# Autodesk Inventor assembly: Intake New Robot
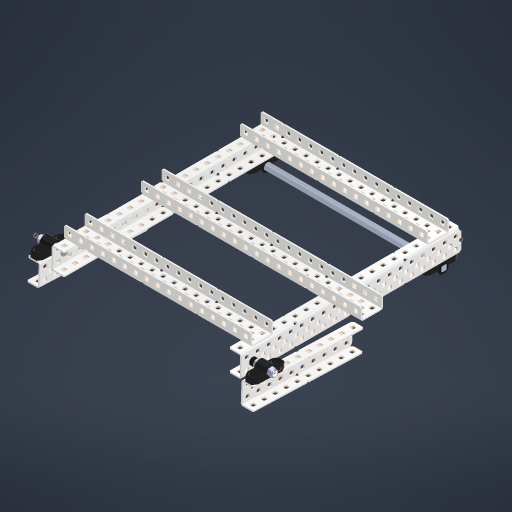
[picture p0: Inventor's stored thumbnail of the model, 512x512]
Saved by Autodesk Inventor 2023 (Build 270158000, 158)
## iProperties
Created: 2023-11-27
Part Number: Intake New Robot
Document SubType Name: Assembly
Designer: Robodox
Author: Robodox
## Documents named in this file (17)
- C:\Users\diego\OneDrive\Documents\GitHub\2023-599Z\BBotCAD\Intake New Robot.iam
- C:\Users\diego\OneDrive\Documents\GitHub\2023-599Z\BBotCAD\VEX-CAD-Inventor-1.4.0\Structure\C Channel\Aluminum 1x2x1\Alu C 1x2x1x10.ipt
- C:\Users\diego\OneDrive\Documents\GitHub\2023-599Z\BBotCAD\VEX-CAD-Inventor-1.4.0\Structure\Hardware\Screw Steel - Star\SScrew Star Smooth 1.000.ipt
- C:\Users\Robodox\Documents\GitHub\2023-599Z\BBotCAD\VEX-CAD-Inventor-1.4.0\Structure\Hardware\Screw Steel - Star.ipt
- C:\Users\diego\OneDrive\Documents\GitHub\2023-599Z\BBotCAD\VEX-CAD-Inventor-1.4.0\Structure\Hardware\Nut Nylock.ipt
- C:\Users\diego\OneDrive\Documents\GitHub\2023-599Z\BBotCAD\VEX-CAD-Inventor-1.4.0\Structure\Hardware\Nut Keps.ipt
- C:\Users\diego\OneDrive\Documents\GitHub\2023-599Z\BBotCAD\VEX-CAD-Inventor-1.4.0\Motion\Spacers\Spacer Plastic\PSpacer 4.6.ipt
- C:\Users\Robodox\Documents\GitHub\2023-599Z\BBotCAD\VEX-CAD-Inventor-1.4.0\Motion\Spacers\Spacer Plastic.ipt
- C:\Users\diego\OneDrive\Documents\GitHub\2023-599Z\BBotCAD\VEX-CAD-Inventor-1.4.0\Structure\C Channel\Aluminum 1x2x1\Alu C 1x2x1x20.ipt
- C:\Users\diego\OneDrive\Documents\GitHub\2023-599Z\BBotCAD\VEX-CAD-Inventor-1.4.0\Structure\C Channel\Aluminum 1x2x1\Alu C 1x2x1x1.ipt
- C:\Users\diego\OneDrive\Documents\GitHub\2023-599Z\BBotCAD\VEX-CAD-Inventor-1.4.0\Motion\Shaft HS\HS Pillow Bearing Block.ipt
- C:\Users\diego\OneDrive\Documents\GitHub\2023-599Z\BBotCAD\VEX-CAD-Inventor-1.4.0\Motion\Shaft HS\HS Spacer\HSpacer .0625.ipt
- C:\Users\diego\OneDrive\Documents\GitHub\2023-599Z\BBotCAD\VEX-CAD-Inventor-1.4.0\Motion\Shaft HS\HS Spacer.ipt
- C:\Users\diego\OneDrive\Documents\GitHub\2024-599Z\2024-599Z\Cad\VEX-CAD-Inventor-1.4.0\Structure\C Channel\Aluminum 1x2x1\Alu C 1x2x1x17.ipt
- C:\Users\diego\OneDrive\Documents\GitHub\2024-599Z\2024-599Z\Cad\VEX-CAD-Inventor-1.4.0\Structure\C Channel\Aluminum 1x2x1\Alu C 1x2x1x20.ipt
- C:\Users\diego\OneDrive\Documents\GitHub\2024-599Z\2024-599Z\Cad\VEX-CAD-Inventor-1.4.0\Motion\Shaft HS\Shaft HS\Shaft HS 8.5 in.ipt
- C:\Users\diego\OneDrive\Documents\GitHub\2024-599Z\2024-599Z\Cad\VEX-CAD-Inventor-1.4.0\Motion\Shaft HS\Shaft HS.ipt
## Components (24 placed, 11 different names)
1. Alu C 1x2x1x10:1 — Insert:24, Insert:25
2. Alu C 1x2x1x10:2 — Insert:26, Insert:27
3. SScrew Star Smooth 1.000:1 — Insert:5, Insert:21, Insert:23, Insert:35
4. Nut Nylock:1 — Insert:23
5. Nut Nylock:2 — Insert:15
6. Nut Keps:2 — Insert:13, Mate:5
7. PSpacer 4.6:1 — Insert:21, Insert:22
8. Alu C 1x2x1x20:2 — Insert:5, Insert:30, Insert:33, Insert:37, Insert:38, Insert:40, Mate:16, Insert:42, Insert:43
9. Nut Keps:3 — Insert:22
10. Alu C 1x2x1x1:1 — Insert:14, Mate:4
11. Alu C 1x2x1x20:4 — Insert:11, Insert:12, Insert:29, Insert:34, Insert:36, Insert:39, Insert:41, Insert:44
12. SScrew Star Smooth 1.000:2 — Insert:11, Insert:14, Insert:15
13. PSpacer 4.6:2 — Insert:12, Insert:13
14. HS Pillow Bearing Block:1 — Insert:26, Insert:27, Mate:4, Mate:5
15. HS Pillow Bearing Block:2 — Insert:24, Insert:25, Mate:14, Mate:15
16. HS Pillow Bearing Block:3 — Insert:30, Insert:33, Mate:18
17. HS Pillow Bearing Block:4 — Insert:29, Insert:34
18. HSpacer .0625:1 — Insert:47, Mate:18
19. Alu C 1x2x1x1:2 — Insert:35, Mate:14, Mate:15
20. Alu C 1x2x1x17:1 — Insert:36, Insert:37, Insert:38, Insert:39
21. Alu C 1x2x1x17:2 — Insert:40, Insert:41
22. HSpacer .0625:2 — Insert:46
23. Alu C 1x2x1x20:5 — Mate:16, Insert:42, Insert:43, Insert:44
24. Shaft HS 8.5 in:1 — Insert:46, Insert:47
## Relationships (35: Insert 29, Mate 6)
- Insert:5: SScrew Star Smooth 1.000:1 ↔ Alu C 1x2x1x20:2
- Insert:11: Alu C 1x2x1x20:4 ↔ SScrew Star Smooth 1.000:2
- Insert:12: Alu C 1x2x1x20:4 ↔ PSpacer 4.6:2
- Insert:13: Nut Keps:2 ↔ PSpacer 4.6:2
- Insert:14 (-15.494 mm): Alu C 1x2x1x1:1 ↔ SScrew Star Smooth 1.000:2
- Insert:15 (-3.048 mm): Nut Nylock:2 ↔ SScrew Star Smooth 1.000:2
- Insert:21 (-23.8252 mm): SScrew Star Smooth 1.000:1 ↔ PSpacer 4.6:1
- Insert:22: PSpacer 4.6:1 ↔ Nut Keps:3
- Insert:23 (-3.048 mm): SScrew Star Smooth 1.000:1 ↔ Nut Nylock:1
- Insert:24: Alu C 1x2x1x10:1 ↔ HS Pillow Bearing Block:2
- Insert:25: Alu C 1x2x1x10:1 ↔ HS Pillow Bearing Block:2
- Insert:26: Alu C 1x2x1x10:2 ↔ HS Pillow Bearing Block:1
- Insert:27: Alu C 1x2x1x10:2 ↔ HS Pillow Bearing Block:1
- Mate:4: Alu C 1x2x1x1:1 ↔ HS Pillow Bearing Block:1
- Mate:5: Nut Keps:2 ↔ HS Pillow Bearing Block:1
- Insert:29: Alu C 1x2x1x20:4 ↔ HS Pillow Bearing Block:4
- Insert:30: Alu C 1x2x1x20:2 ↔ HS Pillow Bearing Block:3
- Insert:33: Alu C 1x2x1x20:2 ↔ HS Pillow Bearing Block:3
- Insert:34: Alu C 1x2x1x20:4 ↔ HS Pillow Bearing Block:4
- Insert:35 (8.382 mm): SScrew Star Smooth 1.000:1 ↔ Alu C 1x2x1x1:2
- Mate:14: HS Pillow Bearing Block:2 ↔ Alu C 1x2x1x1:2
- Mate:15: HS Pillow Bearing Block:2 ↔ Alu C 1x2x1x1:2
- Insert:36: Alu C 1x2x1x20:4 ↔ Alu C 1x2x1x17:1
- Insert:37: Alu C 1x2x1x20:2 ↔ Alu C 1x2x1x17:1
- Insert:38: Alu C 1x2x1x20:2 ↔ Alu C 1x2x1x17:1
- Insert:39: Alu C 1x2x1x20:4 ↔ Alu C 1x2x1x17:1
- Insert:40: Alu C 1x2x1x20:2 ↔ Alu C 1x2x1x17:2
- Insert:41: Alu C 1x2x1x20:4 ↔ Alu C 1x2x1x17:2
- Mate:16: Alu C 1x2x1x20:2 ↔ Alu C 1x2x1x20:5
- Insert:42: Alu C 1x2x1x20:2 ↔ Alu C 1x2x1x20:5
- Insert:43: Alu C 1x2x1x20:2 ↔ Alu C 1x2x1x20:5
- Insert:44: Alu C 1x2x1x20:4 ↔ Alu C 1x2x1x20:5
- Insert:46: HSpacer .0625:2 ↔ Shaft HS 8.5 in:1
- Insert:47: HSpacer .0625:1 ↔ Shaft HS 8.5 in:1
- Mate:18: HS Pillow Bearing Block:3 ↔ HSpacer .0625:1
